# Autodesk Inventor assembly: projekt
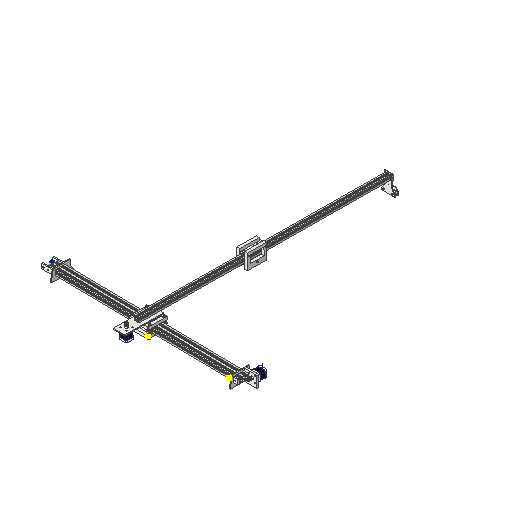
[picture p0: Inventor's stored thumbnail of the model, 512x512]
Saved by Autodesk Inventor 2025.1 (Build 291241000, 241)
## iProperties
Created: 2025-03-27
Part Number: projekt
Document SubType Name: Assembly
Designer: Maciej
Author: Maciej
## Documents named in this file (27)
- C:\Users\Maciej\Desktop\Projekt_przej-ciowy\PP\modele\projekt.iam
- C:\Users\Maciej\Desktop\Projekt_przej-ciowy\PP\modele\MASCHINENBAU_KITZ_25021000000000\25_02_1000(00-00-0)(0).ipt
- C:\Users\Maciej\Desktop\Projekt_przej-ciowy\PP\modele\podstawka pod silnik.ipt
- C:\Users\Maciej\Desktop\Projekt_przej-ciowy\PP\modele\podstawa.ipt
- C:\Users\Maciej\Desktop\Projekt_przej-ciowy\PP\modele\podstawka_prowadzaca.ipt
- C:\Users\Maciej\Desktop\Projekt_przej-ciowy\PP\modele\podstawka_prowadzaca_gora.ipt
- C:\Users\Maciej\Desktop\Projekt_przej-ciowy\PP\modele\wheel-for-v-slot-rail-system-1.snapshot.1\Wheel, V-slot Rail 625-2Z Bearing v4\Wheel, V-slot Rail 625-2Z Bearing v4\Wheel, V-slot Rail 625-2Z Bearing v4.iam
- C:\Users\Maciej\Desktop\Projekt_przej-ciowy\PP\modele\mocowanie_kolek.ipt
- C:\Users\Maciej\Desktop\Projekt_przej-ciowy\PP\modele\tuleja.ipt
- C:\Users\Maciej\Documents\Inventor\Content Center Files\R2025\pl-PL\ISO 4033(2)\ISO 4033 - M5 - ISO.ipt
- C:\Users\Maciej\Desktop\Projekt_przej-ciowy\PP\modele\MASCHINENBAU_KITZ_25011300000000\25_01_1300(00-00-0)(0).ipt
- C:\Users\Maciej\Desktop\Projekt_przej-ciowy\PP\modele\MASCHINENBAU_KITZ_25500540\25_50_0540.ipt
- C:\Users\Maciej\Documents\Inventor\Content Center Files\R2025\pl-PL\ISO 1580\ISO 1580 - M3 x 10_.ipt
- C:\Users\Maciej\Desktop\Projekt_przej-ciowy\PP\modele\stepper-motor-107.snapshot.4\Stepper Motor\Stepper Motor\Stepper Motor.ipt
- C:\Users\Maciej\Desktop\Projekt_przej-ciowy\PP\modele\gt2-timing-pulley-20t-10mm-1.snapshot.11\GT2 Timing Pulley 20T 10mm - Bore_5mm\GT2 Timing Pulley 20T 10mm - Bore_5mm\GT2 Timing Pulley 20T 10mm - Bore_5mm.iam
- C:\Users\Maciej\Documents\Inventor\Content Center Files\R2025\pl-PL\ISO 1580\ISO 1580 - M3 x 12_.ipt
- C:\Users\Maciej\Desktop\Projekt_przej-ciowy\PP\modele\mocowanie_kolek_2.ipt
- C:\Users\Maciej\Desktop\Projekt_przej-ciowy\PP\modele\lozysko.iam
- C:\Users\Maciej\Desktop\Projekt_przej-ciowy\PP\modele\tuleja2.ipt
- C:\Users\Maciej\Desktop\Projekt_przej-ciowy\PP\modele\tuleja3.ipt
- C:\Users\Maciej\Desktop\Projekt_przej-ciowy\PP\modele\płytka_prowadzaca_rysik.ipt
- C:\Users\Maciej\Desktop\PP\modele\wheel-for-v-slot-rail-system-1.snapshot.1\Wheel, V-slot Rail 625-2Z Bearing v4\Wheel, V-slot Rail 625-2Z Bearing v4\Wheel, V-slot Rail 625-2Z Bearing v4.iam
- C:\Users\Maciej\Desktop\Projekt_przej-ciowy\PP\modele\równoważnia.ipt
- C:\Users\Maciej\Desktop\Projekt_przej-ciowy\PP\modele\tuleja_dół.ipt
- C:\Users\Maciej\Documents\Inventor\Content Center Files\R2025\pl-PL\ISO 4014(2)\ISO 4014 - M4 x 25 - ISO.ipt
- C:\Users\Maciej\Documents\Inventor\Content Center Files\R2025\pl-PL\ISO 4032(2)\ISO 4032 - M4 - ISO.ipt
- C:\Users\Maciej\Documents\Inventor\Content Center Files\R2025\pl-PL\PN-85 M-82105 B\PN-85_M-82105 - M 4 x 60 - 0,7.ipt
## Components (84 placed, 25 different names)
1. 25_02_1000(00-00-0)(0):1 — Zestawiające:1, Równoległe:1, Zestawiające:2, Zestawiające:3, Zestawiające:4, Zestawiające:5, Równoległe:2, Równoległe:4, Równoległe:5, Równoległe:6, Równoległe:7, Zestawiające:62, Zestawiające:64, Zestawiające:66, Równoległe:13, Zestawiające:68
2. podstawka pod silnik:1 — Zestawiające:1, Równoległe:1, Zestawiające:2, Zestawiające:52, Zestawiające:54, Zestawiające:55, Zestawiające:61, Wstawiające:6, Wstawiające:7, Wstawiające:8, Wstawiające:9, Zestawiające:63, Wstawiające:10, Zestawiające:65, Wstawiające:11
3. podstawa:1 — Zestawiające:3, Zestawiające:4, Zestawiające:67, Zestawiające:69, Wstawiające:12, Wstawiające:13, Zestawiające:70, Równoległe:14, Zestawiające:72, Zestawiające:74, Zestawiające:76, Zestawiające:109, Zestawiające:111
4. podstawka_prowadzaca_gora:1 — Zestawiające:5, Równoległe:2, Zestawiające:6, Równoległe:3, Zestawiające:7, Zestawiające:9, Zestawiające:10, Zestawiające:11, Zestawiające:41, Zestawiające:43, Zestawiające:45, Zestawiające:47, Zestawiające:48, Zestawiające:49, Zestawiające:50, Zestawiające:51, Wstawiające:1, Zestawiające:56, Zestawiające:57, Zestawiające:58, Zestawiające:59, Zestawiające:60, Wstawiające:2, Wstawiające:3, Wstawiające:4, Wstawiające:5
5. podstawka_prowadzaca:1 — Zestawiające:6, Równoległe:3, Zestawiające:7, Zestawiające:8, Zestawiające:12, Równoległe:8, Zestawiające:13, Zestawiające:14, Zestawiające:15, Równoległe:9, Równoległe:10, Równoległe:11, Zestawiające:17, Zestawiające:22, Zestawiające:27, Zestawiające:33, Zestawiające:35, Zestawiające:37, Zestawiające:39
6. Wheel, V-slot Rail 625-2Z Bearing v4:1 [sub-assembly] — Zestawiające:8, Równoległe:4, Zestawiające:25, Zestawiające:29
7. Wheel, V-slot Rail 625-2Z Bearing v4:2 [sub-assembly] — Zestawiające:9, Równoległe:5, Zestawiające:31
8. Wheel, V-slot Rail 625-2Z Bearing v4:3 [sub-assembly] — Zestawiające:10, Równoległe:6, Zestawiające:18
9. Wheel, V-slot Rail 625-2Z Bearing v4:4 [sub-assembly] — Zestawiające:11, Równoległe:7, Zestawiające:20
10. mocowanie_kolek:1 — Zestawiające:12, Równoległe:8, Zestawiające:21, Zestawiające:23, Zestawiające:36, Zestawiające:42
11. mocowanie_kolek:2 — Zestawiające:13, Równoległe:11, Zestawiające:16, Zestawiające:19, Zestawiające:38, Zestawiające:46
12. mocowanie_kolek:3 — Zestawiające:15, Równoległe:10, Zestawiające:24, Zestawiające:28, Zestawiające:32, Zestawiające:44
13. mocowanie_kolek:4 — Zestawiające:14, Równoległe:9, Zestawiające:26, Zestawiające:30, Zestawiające:34, Zestawiające:40
14. tuleja:1 — Zestawiające:16, Zestawiające:17
15. tuleja:2 — Zestawiające:18, Zestawiające:19
16. tuleja:3 — Zestawiające:20, Zestawiające:21
17. tuleja:4 — Zestawiające:22, Zestawiające:23
18. tuleja:5 — Zestawiające:30, Zestawiające:31
19. tuleja:6 — Zestawiające:28, Zestawiające:29
20. tuleja:7 — Zestawiające:26, Zestawiające:27
21. tuleja:8 — Zestawiające:24, Zestawiające:25
22. ISO 4033 M5:1 — Zestawiające:32, Zestawiające:33
23. ISO 4033 M5:2 — Zestawiające:34, Zestawiające:35
24. ISO 4033 M5:3 — Zestawiające:36, Zestawiające:37
25. ISO 4033 M5:4 — Zestawiające:38, Zestawiające:39
26. ISO 4033 M5:5 — Zestawiające:40, Zestawiające:41
27. ISO 4033 M5:6 — Zestawiające:42, Zestawiające:43
28. ISO 4033 M5:7 — Zestawiające:44, Zestawiające:45
29. ISO 4033 M5:8 — Zestawiające:46, Zestawiające:47
30. 25_01_1300(00-00-0)(0):1 — Zestawiające:48, Zestawiające:49, Równoległe:12, Zestawiające:77, Zestawiające:78, Równoległe:15, Zestawiające:85, Zestawiające:86, Równoległe:18, Zestawiające:104, Zestawiające:106, Zestawiające:107
31. 25_50_0540:1 — Zestawiające:50, Zestawiające:51, Równoległe:12
32. ISO 1580 M3 x 10:1 — Wstawiające:1
33. Stepper Motor:1 — Zestawiające:52, Zestawiające:53, Zestawiające:55, Zestawiające:61
34. GT2 Timing Pulley 20T 10mm - Bore_5mm:1 [sub-assembly] — Zestawiające:56, Zestawiające:57
35. GT2 Timing Pulley 20T 10mm - Bore_5mm:2 [sub-assembly] — Zestawiające:53, Zestawiające:54
36. Stepper Motor:2 — Zestawiające:58, Zestawiające:59, Zestawiające:60
37. ISO 1580 M3 x 12:1 — Wstawiające:2
38. ISO 1580 M3 x 12:2 — Wstawiające:3
39. ISO 1580 M3 x 12:3 — Wstawiające:4
40. ISO 1580 M3 x 12:4 — Wstawiające:5
41. ISO 1580 M3 x 12:5 — Wstawiające:6
42. ISO 1580 M3 x 12:6 — Wstawiające:7
43. ISO 1580 M3 x 12:7 — Wstawiające:8
44. ISO 1580 M3 x 12:8 — Wstawiające:9
45. 25_50_0540:2 — Zestawiające:62, Zestawiające:63
46. ISO 1580 M3 x 12:9 — Wstawiające:10
47. 25_50_0540:3 — Zestawiające:64, Zestawiające:65
48. ISO 1580 M3 x 12:10 — Wstawiające:11
49. 25_50_0540:4 — Zestawiające:66, Zestawiające:67, Równoległe:13
50. 25_50_0540:5 — Zestawiające:68, Zestawiające:69
51. ISO 1580 M3 x 12:11 — Wstawiające:12
52. ISO 1580 M3 x 12:12 — Wstawiające:13
53. mocowanie_kolek_2:1 — Zestawiające:70, Równoległe:14, Zestawiające:71, Zestawiające:73, Zestawiające:75, Zestawiające:108, Zestawiające:110
54. lozysko:1 [sub-assembly] — Zestawiające:71, Zestawiające:72
55. tuleja2:1 — Zestawiające:73, Zestawiające:74
56. tuleja3:1 — Zestawiające:75, Zestawiające:76
57. płytka_prowadzaca_rysik:1 — Zestawiające:77, Równoległe:15, Równoległe:16, Równoległe:17, Zestawiające:79, Zestawiające:80, Wstawiające:21, Zestawiające:113, Wstawiające:22
58. płytka_prowadzaca_rysik:2 — Zestawiające:78, Równoległe:16, Równoległe:17, Zestawiające:81, Zestawiające:82, Zestawiające:83, Zestawiające:84, Wstawiające:18, Wstawiające:19, Wstawiające:20
59. Wheel, V-slot Rail 625-2Z Bearing v4:5 [sub-assembly] — Zestawiające:81, Zestawiające:84
60. Wheel, V-slot Rail 625-2Z Bearing v4:6 [sub-assembly] — Zestawiające:79, Zestawiające:82
61. Wheel, V-slot Rail 625-2Z Bearing v4:7 [sub-assembly] — Zestawiające:80, Zestawiające:83
62. równoważnia:1 — Zestawiające:85, Zestawiające:86, Równoległe:18, Zestawiające:87, Zestawiające:88, Zestawiające:89, Zestawiające:90, Zestawiające:91, Zestawiające:92, Zestawiające:93, Zestawiające:94, Wstawiające:14, Wstawiające:15, Zestawiające:100, Zestawiające:102, Zestawiające:103, Zestawiające:105, Wstawiające:16, Wstawiające:17
63. Wheel, V-slot Rail 625-2Z Bearing v4:8 [sub-assembly] — Zestawiające:95, Zestawiające:96
64. Wheel, V-slot Rail 625-2Z Bearing v4:9 [sub-assembly] — Zestawiające:97, Zestawiające:98
65. tuleja_dół:1 — Zestawiające:87, Zestawiające:94, Zestawiające:96
66. tuleja_dół:2 — Zestawiające:88, Zestawiające:93
67. tuleja_dół:3 — Zestawiające:89, Zestawiające:92
68. tuleja_dół:4 — Zestawiające:90, Zestawiające:91, Zestawiające:98
69. ISO 4014 M4 x 25:1 — Wstawiające:14, Zestawiające:95, Zestawiające:99
70. ISO 4014 M4 x 25:2 — Wstawiające:15, Zestawiające:97, Zestawiające:101
71. ISO 4032 M4:1 — Zestawiające:99, Zestawiające:100
72. ISO 4032 M4:2 — Zestawiające:101, Zestawiające:102
73. 25_50_0540:6 — Zestawiające:103, Zestawiające:104
74. 25_50_0540:7 — Zestawiające:105, Zestawiające:106, Zestawiające:107
75. ISO 1580 M3 x 12:13 — Wstawiające:16
76. ISO 1580 M3 x 12:14 — Wstawiające:17
77. ISO 4032 M4:3 — Zestawiające:108, Zestawiające:109
78. ISO 4032 M4:4 — Zestawiające:110, Zestawiające:111
79. PN-85/M-82105 Klasa B M 4 x 60:1 — Wstawiające:18, Zestawiające:112
80. PN-85/M-82105 Klasa B M 4 x 60:2 — Wstawiające:19
81. PN-85/M-82105 Klasa B M 4 x 60:3 — Wstawiające:20
82. ISO 4032 M4:5 — Wstawiające:21
83. ISO 4032 M4:6 — Zestawiające:112, Zestawiające:113
84. ISO 4032 M4:7 — Wstawiające:22
## Relationships (153: Mate 113, Insert 22, Flush 18)
- Zestawiające:1 [Mate]: 25_02_1000(00-00-0)(0):1 ↔ podstawka pod silnik:1
- Równoległe:1 [Flush]: 25_02_1000(00-00-0)(0):1 ↔ podstawka pod silnik:1
- Zestawiające:2 [Mate]: 25_02_1000(00-00-0)(0):1 ↔ podstawka pod silnik:1
- Zestawiające:3 [Mate]: 25_02_1000(00-00-0)(0):1 ↔ podstawa:1
- Zestawiające:4 [Mate]: 25_02_1000(00-00-0)(0):1 ↔ podstawa:1
- Zestawiające:5 [Mate]: 25_02_1000(00-00-0)(0):1 ↔ podstawka_prowadzaca_gora:1
- Równoległe:2 [Flush] (-25 mm): 25_02_1000(00-00-0)(0):1 ↔ podstawka_prowadzaca_gora:1
- Zestawiające:6 [Mate] (25 mm): podstawka_prowadzaca_gora:1 ↔ podstawka_prowadzaca:1
- Równoległe:3 [Flush]: podstawka_prowadzaca_gora:1 ↔ podstawka_prowadzaca:1
- Zestawiające:7 [Mate]: podstawka_prowadzaca_gora:1 ↔ podstawka_prowadzaca:1
- Zestawiające:8 [Mate]: podstawka_prowadzaca:1 ↔ Wheel, V-slot Rail 625-2Z Bearing v4:1
- Równoległe:4 [Flush] (6.95 mm): 25_02_1000(00-00-0)(0):1 ↔ Wheel, V-slot Rail 625-2Z Bearing v4:1
- Zestawiające:9 [Mate]: podstawka_prowadzaca_gora:1 ↔ Wheel, V-slot Rail 625-2Z Bearing v4:2
- Zestawiające:10 [Mate]: podstawka_prowadzaca_gora:1 ↔ Wheel, V-slot Rail 625-2Z Bearing v4:3
- Zestawiające:11 [Mate]: podstawka_prowadzaca_gora:1 ↔ Wheel, V-slot Rail 625-2Z Bearing v4:4
- Równoległe:5 [Flush] (6.95 mm): 25_02_1000(00-00-0)(0):1 ↔ Wheel, V-slot Rail 625-2Z Bearing v4:2
- Równoległe:6 [Flush] (6.95 mm): 25_02_1000(00-00-0)(0):1 ↔ Wheel, V-slot Rail 625-2Z Bearing v4:3
- Równoległe:7 [Flush] (6.95 mm): 25_02_1000(00-00-0)(0):1 ↔ Wheel, V-slot Rail 625-2Z Bearing v4:4
- Zestawiające:12 [Mate]: podstawka_prowadzaca:1 ↔ mocowanie_kolek:1
- Równoległe:8 [Flush] (-7.5 mm): podstawka_prowadzaca:1 ↔ mocowanie_kolek:1
- Zestawiające:13 [Mate]: podstawka_prowadzaca:1 ↔ mocowanie_kolek:2
- Zestawiające:14 [Mate]: podstawka_prowadzaca:1 ↔ mocowanie_kolek:4
- Zestawiające:15 [Mate]: podstawka_prowadzaca:1 ↔ mocowanie_kolek:3
- Równoległe:9 [Flush] (-7.5 mm): podstawka_prowadzaca:1 ↔ mocowanie_kolek:4
- Równoległe:10 [Flush] (-7.5 mm): podstawka_prowadzaca:1 ↔ mocowanie_kolek:3
- Równoległe:11 [Flush] (-7.5 mm): podstawka_prowadzaca:1 ↔ mocowanie_kolek:2
- Zestawiające:16 [Mate]: mocowanie_kolek:2 ↔ tuleja:1
- Zestawiające:17 [Mate]: podstawka_prowadzaca:1 ↔ tuleja:1
- Zestawiające:18 [Mate]: Wheel, V-slot Rail 625-2Z Bearing v4:3 ↔ tuleja:2
- Zestawiające:19 [Mate]: mocowanie_kolek:2 ↔ tuleja:2
- Zestawiające:20 [Mate]: Wheel, V-slot Rail 625-2Z Bearing v4:4 ↔ tuleja:3
- Zestawiające:21 [Mate]: mocowanie_kolek:1 ↔ tuleja:3
- Zestawiające:22 [Mate]: podstawka_prowadzaca:1 ↔ tuleja:4
- Zestawiające:23 [Mate]: mocowanie_kolek:1 ↔ tuleja:4
- Zestawiające:24 [Mate]: mocowanie_kolek:3 ↔ tuleja:8
- Zestawiające:25 [Mate]: Wheel, V-slot Rail 625-2Z Bearing v4:1 ↔ tuleja:8
- Zestawiające:26 [Mate]: mocowanie_kolek:4 ↔ tuleja:7
- Zestawiające:27 [Mate]: podstawka_prowadzaca:1 ↔ tuleja:7
- Zestawiające:28 [Mate]: mocowanie_kolek:3 ↔ tuleja:6
- Zestawiające:29 [Mate]: Wheel, V-slot Rail 625-2Z Bearing v4:1 ↔ tuleja:6
- Zestawiające:30 [Mate]: mocowanie_kolek:4 ↔ tuleja:5
- Zestawiające:31 [Mate]: Wheel, V-slot Rail 625-2Z Bearing v4:2 ↔ tuleja:5
- Zestawiające:32 [Mate]: mocowanie_kolek:3 ↔ ISO 4033 M5:1
- Zestawiające:33 [Mate]: podstawka_prowadzaca:1 ↔ ISO 4033 M5:1
- Zestawiające:34 [Mate]: mocowanie_kolek:4 ↔ ISO 4033 M5:2
- Zestawiające:35 [Mate]: podstawka_prowadzaca:1 ↔ ISO 4033 M5:2
- Zestawiające:36 [Mate]: mocowanie_kolek:1 ↔ ISO 4033 M5:3
- Zestawiające:37 [Mate]: podstawka_prowadzaca:1 ↔ ISO 4033 M5:3
- Zestawiające:38 [Mate]: mocowanie_kolek:2 ↔ ISO 4033 M5:4
- Zestawiające:39 [Mate]: podstawka_prowadzaca:1 ↔ ISO 4033 M5:4
- Zestawiające:40 [Mate]: mocowanie_kolek:4 ↔ ISO 4033 M5:5
- Zestawiające:41 [Mate]: podstawka_prowadzaca_gora:1 ↔ ISO 4033 M5:5
- Zestawiające:42 [Mate]: mocowanie_kolek:1 ↔ ISO 4033 M5:6
- Zestawiające:43 [Mate]: podstawka_prowadzaca_gora:1 ↔ ISO 4033 M5:6
- Zestawiające:44 [Mate]: mocowanie_kolek:3 ↔ ISO 4033 M5:7
- Zestawiające:45 [Mate]: podstawka_prowadzaca_gora:1 ↔ ISO 4033 M5:7
- Zestawiające:46 [Mate]: mocowanie_kolek:2 ↔ ISO 4033 M5:8
- Zestawiające:47 [Mate]: podstawka_prowadzaca_gora:1 ↔ ISO 4033 M5:8
- Zestawiające:48 [Mate]: podstawka_prowadzaca_gora:1 ↔ 25_01_1300(00-00-0)(0):1
- Zestawiające:49 [Mate]: podstawka_prowadzaca_gora:1 ↔ 25_01_1300(00-00-0)(0):1
- Zestawiające:50 [Mate] (2 mm): podstawka_prowadzaca_gora:1 ↔ 25_50_0540:1
- Zestawiające:51 [Mate]: podstawka_prowadzaca_gora:1 ↔ 25_50_0540:1
- Wstawiające:1 [Insert]: podstawka_prowadzaca_gora:1 ↔ ISO 1580 M3 x 10:1
- Równoległe:12 [Flush]: 25_01_1300(00-00-0)(0):1 ↔ 25_50_0540:1
- Zestawiające:52 [Mate]: podstawka pod silnik:1 ↔ Stepper Motor:1
- Zestawiające:53 [Mate]: Stepper Motor:1 ↔ GT2 Timing Pulley 20T 10mm - Bore_5mm:2
- Zestawiające:54 [Mate] (1 mm): podstawka pod silnik:1 ↔ GT2 Timing Pulley 20T 10mm - Bore_5mm:2
- Zestawiające:55 [Mate]: podstawka pod silnik:1 ↔ Stepper Motor:1
- Zestawiające:56 [Mate]: podstawka_prowadzaca_gora:1 ↔ GT2 Timing Pulley 20T 10mm - Bore_5mm:1
- Zestawiające:57 [Mate] (1 mm): podstawka_prowadzaca_gora:1 ↔ GT2 Timing Pulley 20T 10mm - Bore_5mm:1
- Zestawiające:58 [Mate]: podstawka_prowadzaca_gora:1 ↔ Stepper Motor:2
- Zestawiające:59 [Mate]: podstawka_prowadzaca_gora:1 ↔ Stepper Motor:2
- Zestawiające:60 [Mate]: podstawka_prowadzaca_gora:1 ↔ Stepper Motor:2
- Wstawiające:2 [Insert]: podstawka_prowadzaca_gora:1 ↔ ISO 1580 M3 x 12:1
- Wstawiające:3 [Insert]: podstawka_prowadzaca_gora:1 ↔ ISO 1580 M3 x 12:2
- Wstawiające:4 [Insert]: podstawka_prowadzaca_gora:1 ↔ ISO 1580 M3 x 12:3
- Wstawiające:5 [Insert]: podstawka_prowadzaca_gora:1 ↔ ISO 1580 M3 x 12:4
- Zestawiające:61 [Mate]: podstawka pod silnik:1 ↔ Stepper Motor:1
- Wstawiające:6 [Insert]: podstawka pod silnik:1 ↔ ISO 1580 M3 x 12:5
- Wstawiające:7 [Insert]: podstawka pod silnik:1 ↔ ISO 1580 M3 x 12:6
- Wstawiające:8 [Insert]: podstawka pod silnik:1 ↔ ISO 1580 M3 x 12:7
- Wstawiające:9 [Insert]: podstawka pod silnik:1 ↔ ISO 1580 M3 x 12:8
- Zestawiające:62 [Mate]: 25_02_1000(00-00-0)(0):1 ↔ 25_50_0540:2
- Zestawiające:63 [Mate]: podstawka pod silnik:1 ↔ 25_50_0540:2
- Wstawiające:10 [Insert]: podstawka pod silnik:1 ↔ ISO 1580 M3 x 12:9
- Zestawiające:64 [Mate]: 25_02_1000(00-00-0)(0):1 ↔ 25_50_0540:3
- Zestawiające:65 [Mate]: podstawka pod silnik:1 ↔ 25_50_0540:3
- Wstawiające:11 [Insert]: podstawka pod silnik:1 ↔ ISO 1580 M3 x 12:10
- Zestawiające:66 [Mate]: 25_02_1000(00-00-0)(0):1 ↔ 25_50_0540:4
- Zestawiające:67 [Mate]: podstawa:1 ↔ 25_50_0540:4
- Równoległe:13 [Flush]: 25_02_1000(00-00-0)(0):1 ↔ 25_50_0540:4
- Zestawiające:68 [Mate]: 25_02_1000(00-00-0)(0):1 ↔ 25_50_0540:5
- Zestawiające:69 [Mate]: podstawa:1 ↔ 25_50_0540:5
- Wstawiające:12 [Insert]: podstawa:1 ↔ ISO 1580 M3 x 12:11
- Wstawiające:13 [Insert]: podstawa:1 ↔ ISO 1580 M3 x 12:12
- Zestawiające:70 [Mate]: podstawa:1 ↔ mocowanie_kolek_2:1
- Równoległe:14 [Flush] (4 mm): podstawa:1 ↔ mocowanie_kolek_2:1
- Zestawiające:71 [Mate]: mocowanie_kolek_2:1 ↔ lozysko:1
- Zestawiające:72 [Mate] (8.35 mm): podstawa:1 ↔ lozysko:1
- Zestawiające:73 [Mate]: mocowanie_kolek_2:1 ↔ tuleja2:1
- Zestawiające:74 [Mate]: podstawa:1 ↔ tuleja2:1
- Zestawiające:75 [Mate]: mocowanie_kolek_2:1 ↔ tuleja3:1
- Zestawiające:76 [Mate]: podstawa:1 ↔ tuleja3:1
- Zestawiające:77 [Mate]: 25_01_1300(00-00-0)(0):1 ↔ płytka_prowadzaca_rysik:1
- Zestawiające:78 [Mate]: 25_01_1300(00-00-0)(0):1 ↔ płytka_prowadzaca_rysik:2
- Równoległe:15 [Flush]: 25_01_1300(00-00-0)(0):1 ↔ płytka_prowadzaca_rysik:1
- Równoległe:16 [Flush]: płytka_prowadzaca_rysik:1 ↔ płytka_prowadzaca_rysik:2
- Równoległe:17 [Flush]: płytka_prowadzaca_rysik:1 ↔ płytka_prowadzaca_rysik:2
- Zestawiające:79 [Mate]: płytka_prowadzaca_rysik:1 ↔ Wheel, V-slot Rail 625-2Z Bearing v4:6
- Zestawiające:80 [Mate]: płytka_prowadzaca_rysik:1 ↔ Wheel, V-slot Rail 625-2Z Bearing v4:7
- Zestawiające:81 [Mate]: płytka_prowadzaca_rysik:2 ↔ Wheel, V-slot Rail 625-2Z Bearing v4:5
- Zestawiające:82 [Mate] (7.4 mm): płytka_prowadzaca_rysik:2 ↔ Wheel, V-slot Rail 625-2Z Bearing v4:6
- Zestawiające:83 [Mate] (7.4 mm): płytka_prowadzaca_rysik:2 ↔ Wheel, V-slot Rail 625-2Z Bearing v4:7
- Zestawiające:84 [Mate] (7.4 mm): płytka_prowadzaca_rysik:2 ↔ Wheel, V-slot Rail 625-2Z Bearing v4:5
- Zestawiające:85 [Mate]: 25_01_1300(00-00-0)(0):1 ↔ równoważnia:1
- Zestawiające:86 [Mate]: 25_01_1300(00-00-0)(0):1 ↔ równoważnia:1
- Równoległe:18 [Flush] (1.76 mm): 25_01_1300(00-00-0)(0):1 ↔ równoważnia:1
- Zestawiające:87 [Mate]: równoważnia:1 ↔ tuleja_dół:1
- Zestawiające:88 [Mate]: równoważnia:1 ↔ tuleja_dół:2
- Zestawiające:89 [Mate]: równoważnia:1 ↔ tuleja_dół:3
- Zestawiające:90 [Mate]: równoważnia:1 ↔ tuleja_dół:4
- Zestawiające:91 [Mate]: równoważnia:1 ↔ tuleja_dół:4
- Zestawiające:92 [Mate]: równoważnia:1 ↔ tuleja_dół:3
- Zestawiające:93 [Mate]: równoważnia:1 ↔ tuleja_dół:2
- Zestawiające:94 [Mate]: równoważnia:1 ↔ tuleja_dół:1
- Wstawiające:14 [Insert]: równoważnia:1 ↔ ISO 4014 M4 x 25:1
- Wstawiające:15 [Insert]: równoważnia:1 ↔ ISO 4014 M4 x 25:2
- Zestawiające:95 [Mate]: Wheel, V-slot Rail 625-2Z Bearing v4:8 ↔ ISO 4014 M4 x 25:1
- Zestawiające:96 [Mate]: Wheel, V-slot Rail 625-2Z Bearing v4:8 ↔ tuleja_dół:1
- Zestawiające:97 [Mate]: Wheel, V-slot Rail 625-2Z Bearing v4:9 ↔ ISO 4014 M4 x 25:2
- Zestawiające:98 [Mate]: Wheel, V-slot Rail 625-2Z Bearing v4:9 ↔ tuleja_dół:4
- Zestawiające:99 [Mate]: ISO 4014 M4 x 25:1 ↔ ISO 4032 M4:1
- Zestawiające:100 [Mate]: równoważnia:1 ↔ ISO 4032 M4:1
- Zestawiające:101 [Mate]: ISO 4014 M4 x 25:2 ↔ ISO 4032 M4:2
- Zestawiające:102 [Mate]: równoważnia:1 ↔ ISO 4032 M4:2
- Zestawiające:103 [Mate]: równoważnia:1 ↔ 25_50_0540:6
- Zestawiające:104 [Mate]: 25_01_1300(00-00-0)(0):1 ↔ 25_50_0540:6
- Zestawiające:105 [Mate]: równoważnia:1 ↔ 25_50_0540:7
- Zestawiające:106 [Mate]: 25_01_1300(00-00-0)(0):1 ↔ 25_50_0540:7
- Zestawiające:107 [Mate] (0.25 mm): 25_01_1300(00-00-0)(0):1 ↔ 25_50_0540:7
- Wstawiające:16 [Insert]: równoważnia:1 ↔ ISO 1580 M3 x 12:13
- Wstawiające:17 [Insert]: równoważnia:1 ↔ ISO 1580 M3 x 12:14
- Zestawiające:108 [Mate]: mocowanie_kolek_2:1 ↔ ISO 4032 M4:3
- Zestawiające:109 [Mate]: podstawa:1 ↔ ISO 4032 M4:3
- Zestawiające:110 [Mate]: mocowanie_kolek_2:1 ↔ ISO 4032 M4:4
- Zestawiające:111 [Mate]: podstawa:1 ↔ ISO 4032 M4:4
- Wstawiające:18 [Insert]: płytka_prowadzaca_rysik:2 ↔ PN-85/M-82105 Klasa B M 4 x 60:1
- Wstawiające:19 [Insert]: płytka_prowadzaca_rysik:2 ↔ PN-85/M-82105 Klasa B M 4 x 60:2
- Wstawiające:20 [Insert]: płytka_prowadzaca_rysik:2 ↔ PN-85/M-82105 Klasa B M 4 x 60:3
- Wstawiające:21 [Insert]: płytka_prowadzaca_rysik:1 ↔ ISO 4032 M4:5
- Zestawiające:112 [Mate]: PN-85/M-82105 Klasa B M 4 x 60:1 ↔ ISO 4032 M4:6
- Zestawiające:113 [Mate]: płytka_prowadzaca_rysik:1 ↔ ISO 4032 M4:6
- Wstawiające:22 [Insert]: płytka_prowadzaca_rysik:1 ↔ ISO 4032 M4:7
